# Autodesk Inventor assembly: Rb oven housing
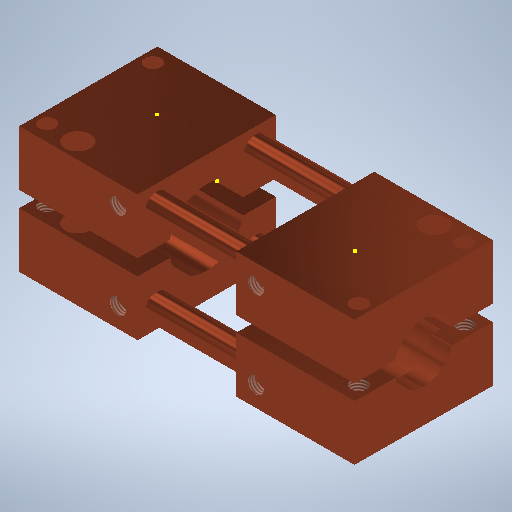
[picture p0: Inventor's stored thumbnail of the model, 512x512]
Saved by Autodesk Inventor 2025.3 (Build 293356000, 356)
## iProperties
Created: 2025-04-24
Part Number: Rb oven housing
Document SubType Name: Assembly
Designer: E. Moreno
Author: E. Moreno
Title: Carcasa Horno - Ensamblado
## Documents named in this file (3)
- E:\Users\USER\Documents\GitHub\LAFriOC\Rb oven\Rb oven housing\Modificación\Rb oven housing.iam
- E:\Users\USER\Documents\GitHub\LAFriOC\Rb oven\Rb oven housing\Modificación\Rb oven housing - Bottom.iam
- E:\Users\USER\Documents\GitHub\LAFriOC\Rb oven\Rb oven housing\Modificación\Rb oven housing - Top.iam
## Components (2 placed, 2 different names)
1. Rb oven housing - Bottom:1 [sub-assembly] — Mate:1, Mate:2
2. Rb oven housing - Top:1 [sub-assembly] — Mate:1, Mate:2
## Relationships (2: Mate 2)
- Mate:1 (18 mm): Rb oven housing - Bottom:1 ↔ Rb oven housing - Top:1
- Mate:2: Rb oven housing - Bottom:1 ↔ Rb oven housing - Top:1
